# Autodesk Inventor assembly: Body V7 Pi5 - Removable Electronics
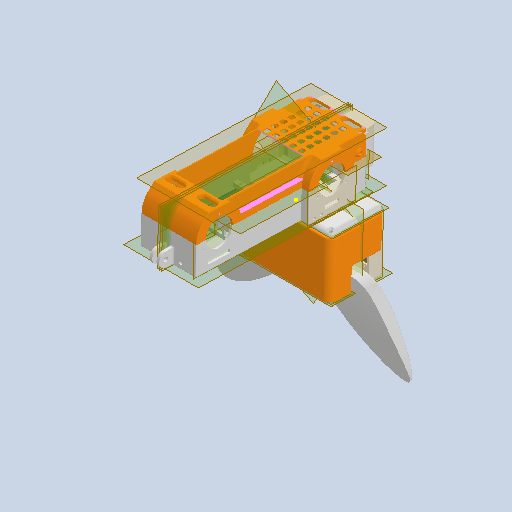
[picture p0: Inventor's stored thumbnail of the model, 512x512]
Saved by Autodesk Inventor 2024.2 (Build 282272000, 272)
## iProperties
Created: 2025-09-19
Part Number: Body V7 Pi5 - Removable Electronics
Document SubType Name: Assembly
Designer: AdminForWorker
Title: Body V7 Pi5 - Removable Electronics v36
Author: AdminForWorker
## Documents named in this file (20)
- D:\dog\fox\construction\fox\body\тело лисы.iam
- D:\dog\fox\construction\fox\boards\3D_PCB4_2024-01-15 v3.iam
- D:\dog\fox\construction\fox\legs\Part222.ipt
- D:\dog\fox\construction\fox\body\верхняя часть.ipt
- D:\dog\fox\construction\fox\body\крышка камера.ipt
- D:\dog\fox\construction\fox\body\спина.ipt
- D:\dog\fox\construction\fox\body\шея.ipt
- D:\dog\fox\construction\fox\body\лицо.ipt
- D:\dog\fox\construction\fox\body\голова потолок.ipt
- D:\dog\fox\construction\fox\body\ухо правое.ipt
- D:\dog\fox\construction\fox\raspberry\0329_экран.ipt
- D:\dog\fox\construction\fox\body\JX Servo PDI-HV2006MG.ipt
- D:\dog\fox\construction\fox\body\накладка.ipt
- D:\dog\fox\construction\fox\boards\плата управления\плата управления.iam
- D:\dog\fox\construction\fox\boards\динамик\динамик.ipt
- D:\dog\fox\construction\3dstep\крепление сервоприводов.ipt
- D:\dog\fox\construction\3dstep\втавки в уши.ipt
- D:\dog\fox\construction\fox\body\крутилка3\крутилка3.ipt
- D:\dog\fox\construction\fox\raspberry\RPiAIHATPlusBoard\RPiAIHATPlusBoard.ipt
- D:\dog\fox\construction\fox\raspberry\RASPBERRY_PI_5\RASPBERRY_PI_5.ipt
## Components (21 placed, 19 different names)
1. плата питания [sub-assembly] — Совмещение:3, Совмещение:4, Совмещение:5
2. крышка камера:1 — Совмещение:14, Совмещение:20
3. основа тела — Заподлицо:1, Заподлицо:2, Заподлицо:3, Заподлицо:13
4. верхняя часть:1 — Заподлицо:1, Заподлицо:2, Заподлицо:3, Совмещение:3, Совмещение:4, Совмещение:5, Заподлицо:14, Заподлицо:16, Заподлицо:17, Заподлицо:18, Совмещение:20
5. потолок — Заподлицо:13, Заподлицо:14, Заподлицо:16, Заподлицо:17, Заподлицо:18, Заподлицо:19, Заподлицо:20
6. шея:1 — Заподлицо:19, Заподлицо:20
7. лицо:1 — Заподлицо:24, Заподлицо:25, Совмещение:6, Совмещение:7, Заподлицо:28, Совмещение:11, Совмещение:12, Совмещение:13, Заподлицо:29, Заподлицо:30, Заподлицо:31, Заподлицо:32, Совмещение:17, Совмещение:18, Совмещение:19, Заподлицо:37, С поворотом:5
8. голова потолок:1 — Заподлицо:24, Заподлицо:25
9. ухо правое:1 — Заподлицо:26, Заподлицо:27, Заподлицо:38, Заподлицо:39
10. 0329_экран:1 — Совмещение:6, Совмещение:7, Заподлицо:28
11. JX Servo PDI-HV2006MG:1 — Совмещение:17, Совмещение:18, Совмещение:19, Заподлицо:34, Заподлицо:35, С поворотом:4
12. JX Servo PDI-HV2006MG:2 — Совмещение:11, Совмещение:12, Совмещение:13, Заподлицо:36, С поворотом:3
13. накладка:1 — Заподлицо:29, Заподлицо:30, Заподлицо:31, Заподлицо:32
14. плата управления:1 [sub-assembly]
15. динамик:1 — Совмещение:14
16. крепление сервоприводов:1 — Заподлицо:34, Заподлицо:35, Заподлицо:36, Заподлицо:37
17. втавки в уши:1 — Заподлицо:38, Заподлицо:39
18. крутилка3:1 — С поворотом:3
19. крутилка3:2 — С поворотом:4
20. RPiAIHATPlusBoard:1 — Совмещение:21, Совмещение:22
21. RASPBERRY_PI_5:1 — С поворотом:5, Совмещение:21, Совмещение:22
## Relationships (48: Flush 30, Mate 15, RevoluteJoint 3)
- Заподлицо:1 [Flush]: основа тела ↔ верхняя часть:1
- Заподлицо:2 [Flush]: основа тела ↔ верхняя часть:1
- Заподлицо:3 [Flush]: основа тела ↔ верхняя часть:1
- Совмещение:3 [Mate] (-15 mm): плата питания ↔ верхняя часть:1
- Совмещение:4 [Mate]: плата питания ↔ верхняя часть:1
- Совмещение:5 [Mate]: плата питания ↔ верхняя часть:1
- [Flush]: крышка камера:1 ↔ верхняя часть:1
- [Flush]: крышка камера:1 ↔ верхняя часть:1
- [Flush]: крышка камера:1 ↔ верхняя часть:1
- [Flush]: крышка камера:1 ↔ верхняя часть:1
- Заподлицо:13 [Flush]: основа тела ↔ потолок
- Заподлицо:14 [Flush]: верхняя часть:1 ↔ потолок
- Заподлицо:16 [Flush]: верхняя часть:1 ↔ потолок
- Заподлицо:17 [Flush]: верхняя часть:1 ↔ потолок
- Заподлицо:18 [Flush]: верхняя часть:1 ↔ потолок
- Заподлицо:19 [Flush]: потолок ↔ шея:1
- Заподлицо:20 [Flush]: потолок ↔ шея:1
- [Flush]: шея:1 ↔ лицо:1
- Заподлицо:24 [Flush]: лицо:1 ↔ голова потолок:1
- Заподлицо:25 [Flush]: лицо:1 ↔ голова потолок:1
- Заподлицо:26 [Flush]: ухо правое:1
- Заподлицо:27 [Flush]: ухо правое:1
- Совмещение:6 [Mate]: лицо:1 ↔ 0329_экран:1
- Совмещение:7 [Mate]: лицо:1 ↔ 0329_экран:1
- Заподлицо:28 [Flush]: лицо:1 ↔ 0329_экран:1
- Совмещение:11 [Mate] (-2 mm): лицо:1 ↔ JX Servo PDI-HV2006MG:2
- Совмещение:12 [Mate] (65 mm): лицо:1 ↔ JX Servo PDI-HV2006MG:2
- Совмещение:13 [Mate] (30 mm): лицо:1 ↔ JX Servo PDI-HV2006MG:2
- Заподлицо:29 [Flush]: лицо:1 ↔ накладка:1
- Заподлицо:30 [Flush]: лицо:1 ↔ накладка:1
- Заподлицо:31 [Flush]: лицо:1 ↔ накладка:1
- Заподлицо:32 [Flush]: лицо:1 ↔ накладка:1
- Совмещение:14 [Mate]: крышка камера:1 ↔ динамик:1
- Совмещение:17 [Mate] (-1 mm): лицо:1 ↔ JX Servo PDI-HV2006MG:1
- Совмещение:18 [Mate] (37 mm): лицо:1 ↔ JX Servo PDI-HV2006MG:1
- Совмещение:19 [Mate] (30 mm): лицо:1 ↔ JX Servo PDI-HV2006MG:1
- Совмещение:20 [Mate]: крышка камера:1 ↔ верхняя часть:1
- Заподлицо:34 [Flush]: JX Servo PDI-HV2006MG:1 ↔ крепление сервоприводов:1
- Заподлицо:35 [Flush]: JX Servo PDI-HV2006MG:1 ↔ крепление сервоприводов:1
- Заподлицо:36 [Flush]: JX Servo PDI-HV2006MG:2 ↔ крепление сервоприводов:1
- Заподлицо:37 [Flush]: лицо:1 ↔ крепление сервоприводов:1
- Заподлицо:38 [Flush]: ухо правое:1 ↔ втавки в уши:1
- Заподлицо:39 [Flush]: ухо правое:1 ↔ втавки в уши:1
- С поворотом:3 [RevoluteJoint]: JX Servo PDI-HV2006MG:2 ↔ крутилка3:1
- С поворотом:4 [RevoluteJoint]: JX Servo PDI-HV2006MG:1 ↔ крутилка3:2
- С поворотом:5 [RevoluteJoint]: лицо:1 ↔ RASPBERRY_PI_5:1
- Совмещение:21 [Mate] (1 mm): RPiAIHATPlusBoard:1 ↔ RASPBERRY_PI_5:1
- Совмещение:22 [Mate] (0.2 mm): RPiAIHATPlusBoard:1 ↔ RASPBERRY_PI_5:1
## Named parameters: d17_d6 = 0 mm
